# Autodesk Inventor assembly: Assembly4
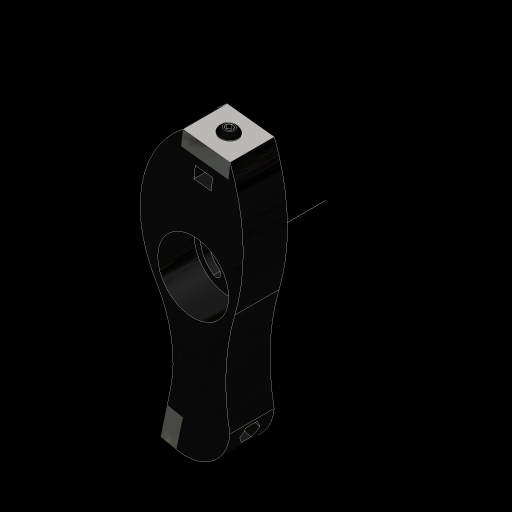
[picture p0: Inventor's stored thumbnail of the model, 512x512]
Saved by Autodesk Inventor 2023 (Build 270158000, 158)
## iProperties
Created: 2023-02-13
Part Number: Assembly4
Document SubType Name: Assembly
Designer: tandu
Mass: 89.4285 g
Surface Area: 172.609 cm^2
Volume: 48.7802 cm^3
Density: 1.8333 g/cm^3
Author: tandu
## Documents named in this file (6)
- C:\Users\tandu\Documents\GrabCAD\Insomnia 2020\Versions\9 Comically Large Weapon 9 28 22\TPUWeapon\TPUWeaponAssembly.iam
- C:\Users\tandu\Documents\GrabCAD\Insomnia 2020\Versions\9 Comically Large Weapon 9 28 22\TPUWeapon\TPUEggBeater.ipt
- C:\Users\tandu\Documents\GrabCAD\Insomnia 2020\Versions\9 Comically Large Weapon 9 28 22\TPUWeapon\Tooth.ipt
- C:\Users\tandu\Documents\GrabCAD\Insomnia 2020\Versions\9 Comically Large Weapon 9 28 22\TPUWeapon\CounterWeight.ipt
- C:\Users\tandu\Documents\GrabCAD\Insomnia 2020\Versions\9 Comically Large Weapon 9 28 22\TPUWeapon\90237A110_High-Strength Steel Nylon-Insert Locknuts.ipt
- C:\Users\tandu\Documents\GrabCAD\Insomnia 2020\Versions\9 Comically Large Weapon 9 28 22\TPUWeapon\16 mm 91239A150_Button Head Hex Drive Screw.ipt
## Components (7 placed, 5 different names)
1. TPUEggBeater:1 — Insert:8, Insert:10, Mate:1, Mate:4, Mate:6, Insert:12, Insert:13, Mate:7, Flush:1
2. Tooth:1 — Insert:13, Flush:1
3. CounterWeight:1 — Insert:12, Mate:7
4. 16 mm 91239A150_Button Head Hex Drive Screw:1
5. 16 mm 91239A150_Button Head Hex Drive Screw:2
6. 90237A110_High-Strength Steel Nylon-Insert Locknuts:2 — Insert:10, Mate:4
7. 90237A110_High-Strength Steel Nylon-Insert Locknuts:5 — Insert:8, Mate:1
## Relationships (11: Insert 6, Mate 4, Flush 1)
- [Insert]: Tooth:1 ↔ 16 mm 91239A150_Button Head Hex Drive Screw:2
- Insert:8: TPUEggBeater:1 ↔ 90237A110_High-Strength Steel Nylon-Insert Locknuts:5
- Insert:10: TPUEggBeater:1 ↔ 90237A110_High-Strength Steel Nylon-Insert Locknuts:2
- Mate:1: TPUEggBeater:1 ↔ 90237A110_High-Strength Steel Nylon-Insert Locknuts:5
- Mate:4: TPUEggBeater:1 ↔ 90237A110_High-Strength Steel Nylon-Insert Locknuts:2
- Mate:6: TPUEggBeater:1
- Insert:12: TPUEggBeater:1 ↔ CounterWeight:1
- Insert:13: TPUEggBeater:1 ↔ Tooth:1
- [Insert]: CounterWeight:1 ↔ 16 mm 91239A150_Button Head Hex Drive Screw:1
- Mate:7: TPUEggBeater:1 ↔ CounterWeight:1
- Flush:1: TPUEggBeater:1 ↔ Tooth:1
